# Autodesk Inventor assembly: peristaltic pump
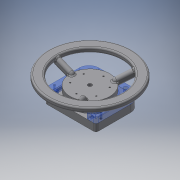
[picture p0: Inventor's stored thumbnail of the model, 180x180]
Saved by Autodesk Inventor 2017 (Build 210142000, 142)
## iProperties
Created: 2018-01-19
Part Number: peristaltic pump
Document SubType Name: Assembly
Designer: RLanting
Author: RLanting
## Documents named in this file (7)
- C:\Users\rmccomber\Documents\st motor\direct drive electronic valving 2\hydraulic steering\steering wheel\peristaltic pump\peristaltic pump.iam
- C:\Users\rmccomber\Documents\st motor\direct drive electronic valving 2\hydraulic steering\steering wheel\peristaltic pump\rotor 2.ipt
- C:\Users\rmccomber\Documents\st motor\direct drive electronic valving 2\hydraulic steering\steering wheel\peristaltic pump\rotor 1.ipt
- C:\Users\rmccomber\Documents\st motor\direct drive electronic valving 2\hydraulic steering\steering wheel\peristaltic pump\608 bearing.ipt
- C:\Users\rmccomber\Documents\st motor\direct drive electronic valving 2\hydraulic steering\steering wheel\peristaltic pump\frame top.ipt
- C:\Users\rmccomber\Documents\st motor\direct drive electronic valving 2\hydraulic steering\steering wheel\peristaltic pump\frame bottom.ipt
- C:\Users\rmccomber\Documents\st motor\direct drive electronic valving 2\hydraulic steering\steering wheel\peristaltic pump\steering wheel.ipt
## Components (11 placed, 6 different names)
1. rotor 2:1 — Mate:1, Mate:2, Mate:3, Mate:4, Mate:5, Mate:6, Mate:7, Mate:8, Mate:9, Mate:10, Mate:11, Mate:12, Mate:13, Mate:14, Mate:15, Mate:17
2. rotor 1:1 — Mate:1, Mate:2, Mate:3, Mate:16, Mate:18, Mate:19
3. 608 bearing:1 — Mate:4, Mate:5
4. 608 bearing:2 — Mate:6, Mate:7
5. 608 bearing:3 — Mate:8, Mate:9
6. 608 bearing:4 — Mate:10, Mate:11
7. 608 bearing:5 — Mate:12, Mate:13
8. 608 bearing:6 — Mate:14, Mate:15
9. frame top:1 — Mate:16, Mate:17, Flush:1, Flush:2
10. frame bottom:1 — Flush:1, Flush:2
11. steering wheel:1 — Mate:18, Mate:19
## Relationships (21: Mate 19, Flush 2)
- Mate:1: rotor 2:1 ↔ rotor 1:1
- Mate:2: rotor 2:1 ↔ rotor 1:1
- Mate:3: rotor 2:1 ↔ rotor 1:1
- Mate:4: rotor 2:1 ↔ 608 bearing:1
- Mate:5: rotor 2:1 ↔ 608 bearing:1
- Mate:6: rotor 2:1 ↔ 608 bearing:2
- Mate:7: rotor 2:1 ↔ 608 bearing:2
- Mate:8: rotor 2:1 ↔ 608 bearing:3
- Mate:9: rotor 2:1 ↔ 608 bearing:3
- Mate:10: rotor 2:1 ↔ 608 bearing:4
- Mate:11: rotor 2:1 ↔ 608 bearing:4
- Mate:12: rotor 2:1 ↔ 608 bearing:5
- Mate:13: rotor 2:1 ↔ 608 bearing:5
- Mate:14: rotor 2:1 ↔ 608 bearing:6
- Mate:15: rotor 2:1 ↔ 608 bearing:6
- Mate:16: rotor 1:1 ↔ frame top:1
- Mate:17: rotor 2:1 ↔ frame top:1
- Flush:1: frame top:1 ↔ frame bottom:1
- Flush:2: frame top:1 ↔ frame bottom:1
- Mate:18: rotor 1:1 ↔ steering wheel:1
- Mate:19: rotor 1:1 ↔ steering wheel:1
